# Autodesk Inventor assembly: Claw2017-18
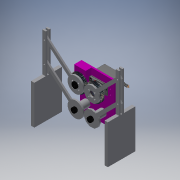
[picture p0: Inventor's stored thumbnail of the model, 180x180]
Saved by Autodesk Inventor 2017 (Build 210142000, 142)
## iProperties
Created: 2017-09-28
Part Number: Claw2017-18
Document SubType Name: Assembly
Designer: User
Author: User
## Documents named in this file (11)
- C:\Robotics\CAD\2017-18_CAD\Claw2017-18.iam
- C:\Robotics\CAD\2017-18_CAD\ClawServoHolder.ipt
- C:\Robotics\CAD\COTSParts\Tetrix\Tetrix servo 180.ipt
- C:\Robotics\CAD\COTSParts\Tetrix\Tetrix Gear 40T.ipt
- C:\Robotics\CAD\COTSParts\Vex\91259A574_ALLOY STEEL SHOULDER SCREW.ipt
- C:\Robotics\CAD\2017-18_CAD\ClawLinkage.ipt
- C:\Robotics\CAD\2017-18_CAD\ClawLinkage - Bottom.ipt
- C:\Robotics\CAD\COTSParts\Vex\91259A541_ALLOY STEEL SHOULDER SCREW.ipt
- C:\Robotics\CAD\2017-18_CAD\0_69inchClawSpacer.ipt
- C:\Robotics\CAD\2017-18_CAD\05incheClawSpacer.ipt
- C:\Robotics\CAD\2017-18_CAD\2BarClawPaddle.ipt
## Components (17 placed, 10 different names)
1. ClawServoHolder:1 — Mate:5, Mate:6, Mate:7, Mate:11, Mate:12, Mate:26, Mate:27, Flush:10, Mate:30, Mate:33
2. Tetrix servo 180:1 — Mate:5, Mate:6, Mate:7, Mate:9, Mate:10
3. Tetrix Gear 40T:1 — Mate:9, Mate:10, Flush:5, Mate:19, Mate:20, Mate:21
4. Tetrix Gear 40T:2 — Mate:11, Mate:12, Flush:5, Mate:13, Mate:14, Mate:22, Mate:23, Mate:24
5. 91259A574_ALLOY STEEL SHOULDER SCREW:1 — Mate:13, Mate:14
6. ClawLinkage:1 — Mate:19, Mate:20, Mate:21, Flush:7, Insert:1
7. ClawLinkage:2 — Mate:22, Mate:23, Mate:24, Flush:8, Mate:42
8. ClawLinkage - Bottom:1 — Flush:8, Mate:27, Mate:28, Mate:41, Mate:43
9. ClawLinkage - Bottom:2 — Flush:7, Mate:26, Mate:31, Mate:39, Insert:2, Mate:44
10. 91259A541_ALLOY STEEL SHOULDER SCREW:1 — Mate:31, Mate:32, Mate:44, Mate:47
11. 91259A541_ALLOY STEEL SHOULDER SCREW:2 — Mate:28, Flush:10, Mate:29, Mate:46
12. 0_69inchClawSpacer:1 — Mate:29, Mate:30, Mate:45
13. 05incheClawSpacer:1 — Mate:47, Mate:48
14. 05incheClawSpacer:2 — Mate:45, Mate:46
15. 0_69inchClawSpacer:2 — Mate:32, Mate:33, Mate:48
16. 2BarClawPaddle:2 — Mate:41, Mate:42, Mate:43
17. 2BarClawPaddle:3 — Mate:39, Insert:1, Insert:2
## Relationships (38: Mate 32, Flush 4, Insert 2)
- Mate:5: ClawServoHolder:1 ↔ Tetrix servo 180:1
- Mate:6: ClawServoHolder:1 ↔ Tetrix servo 180:1
- Mate:7: ClawServoHolder:1 ↔ Tetrix servo 180:1
- Mate:9: Tetrix servo 180:1 ↔ Tetrix Gear 40T:1
- Mate:10: Tetrix servo 180:1 ↔ Tetrix Gear 40T:1
- Mate:11 (1.7526 mm): ClawServoHolder:1 ↔ Tetrix Gear 40T:2
- Mate:12: ClawServoHolder:1 ↔ Tetrix Gear 40T:2
- Flush:5: Tetrix Gear 40T:1 ↔ Tetrix Gear 40T:2
- Mate:13: Tetrix Gear 40T:2 ↔ 91259A574_ALLOY STEEL SHOULDER SCREW:1
- Mate:14: Tetrix Gear 40T:2 ↔ 91259A574_ALLOY STEEL SHOULDER SCREW:1
- Mate:19: Tetrix Gear 40T:1 ↔ ClawLinkage:1
- Mate:20: Tetrix Gear 40T:1 ↔ ClawLinkage:1
- Mate:21: Tetrix Gear 40T:1 ↔ ClawLinkage:1
- Mate:22: Tetrix Gear 40T:2 ↔ ClawLinkage:2
- Mate:23: Tetrix Gear 40T:2 ↔ ClawLinkage:2
- Mate:24: Tetrix Gear 40T:2 ↔ ClawLinkage:2
- Flush:7: ClawLinkage:1 ↔ ClawLinkage - Bottom:2
- Mate:26: ClawServoHolder:1 ↔ ClawLinkage - Bottom:2
- Flush:8: ClawLinkage:2 ↔ ClawLinkage - Bottom:1
- Mate:27: ClawServoHolder:1 ↔ ClawLinkage - Bottom:1
- Mate:28: ClawLinkage - Bottom:1 ↔ 91259A541_ALLOY STEEL SHOULDER SCREW:2
- Flush:10: ClawServoHolder:1 ↔ 91259A541_ALLOY STEEL SHOULDER SCREW:2
- Mate:29: 91259A541_ALLOY STEEL SHOULDER SCREW:2 ↔ 0_69inchClawSpacer:1
- Mate:30: ClawServoHolder:1 ↔ 0_69inchClawSpacer:1
- Mate:31: ClawLinkage - Bottom:2 ↔ 91259A541_ALLOY STEEL SHOULDER SCREW:1
- Mate:32: 91259A541_ALLOY STEEL SHOULDER SCREW:1 ↔ 0_69inchClawSpacer:2
- Mate:33: ClawServoHolder:1 ↔ 0_69inchClawSpacer:2
- Mate:39: ClawLinkage - Bottom:2 ↔ 2BarClawPaddle:3
- Mate:41: ClawLinkage - Bottom:1 ↔ 2BarClawPaddle:2
- Insert:1: ClawLinkage:1 ↔ 2BarClawPaddle:3
- Insert:2: ClawLinkage - Bottom:2 ↔ 2BarClawPaddle:3
- Mate:42: ClawLinkage:2 ↔ 2BarClawPaddle:2
- Mate:43: ClawLinkage - Bottom:1 ↔ 2BarClawPaddle:2
- Mate:44: ClawLinkage - Bottom:2 ↔ 91259A541_ALLOY STEEL SHOULDER SCREW:1
- Mate:45: 0_69inchClawSpacer:1 ↔ 05incheClawSpacer:2
- Mate:46: 91259A541_ALLOY STEEL SHOULDER SCREW:2 ↔ 05incheClawSpacer:2
- Mate:47: 91259A541_ALLOY STEEL SHOULDER SCREW:1 ↔ 05incheClawSpacer:1
- Mate:48: 05incheClawSpacer:1 ↔ 0_69inchClawSpacer:2
